# Autodesk Inventor assembly: Photosensor Assembly Exploded
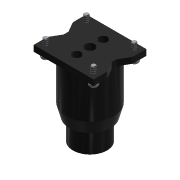
[picture p0: Inventor's stored thumbnail of the model, 180x180]
Saved by Autodesk Inventor 2017 (Build 210142000, 142)
## iProperties
Created: 2016-12-22
Part Number: Photosensor Assembly Exploded
Document SubType Name: Assembly
Designer: ge937963
Author: ge937963
## Documents named in this file (7)
- C:\Users\ge937963\Desktop\Inventor View\Photodiode Assembly.iam
- C:\Users\ge937963\Desktop\Inventor View\Photodiode Holder.ipt
- C:\Users\ge937963\Desktop\Inventor View\Emission Filter Holder.ipt
- C:\Users\ge937963\Desktop\Inventor View\Photodiode Assembly Mount.ipt
- C:\Users\ge937963\Desktop\Inventor View\Photodiode.ipt
- C:\Users\ge937963\Desktop\Inventor View\Screw.ipt
- C:\Users\ge937963\Desktop\Inventor View\Emission Filter.ipt
## Components (13 placed, 6 different names)
1. Photodiode Holder:1 — Mate:15, Mate:16, Mate:18
2. Emission Filter Holder:1 — Mate:18, Mate:19, Mate:21, Mate:22
3. Photodiode Assembly Mount:1 — Mate:16, Mate:20
4. Photodiode:1 — Mate:15
5. Screw:1 — Mate:20
6. Screw:2
7. Screw:3
8. Screw:4 — Mate:19
9. Screw:5
10. Screw:6
11. Screw:7
12. Screw:8
13. Emission Filter:1 — Mate:21, Mate:22
## Relationships (25: Mate 20, Flush 5)
- [Mate]: Photodiode Holder:1 ↔ Emission Filter Holder:1
- [Mate]: Photodiode Holder:1 ↔ Emission Filter Holder:1
- [Mate]: Photodiode Holder:1 ↔ Photodiode Assembly Mount:1
- [Mate]: Photodiode Holder:1 ↔ Photodiode Assembly Mount:1
- [Mate]: Photodiode Holder:1 ↔ Photodiode:1
- [Mate]: Emission Filter Holder:1 ↔ Screw:3
- [Mate]: Emission Filter Holder:1 ↔ Screw:4
- [Flush]: Screw:3 ↔ Screw:4
- [Flush]: Screw:1 ↔ Screw:2
- [Mate]: Photodiode Assembly Mount:1 ↔ Screw:1
- [Mate]: Photodiode Assembly Mount:1 ↔ Screw:2
- [Mate]: Photodiode Assembly Mount:1 ↔ Screw:5
- [Mate]: Photodiode Assembly Mount:1 ↔ Screw:6
- [Mate]: Photodiode Assembly Mount:1 ↔ Screw:7
- [Mate]: Photodiode Assembly Mount:1 ↔ Screw:8
- [Flush]: Screw:7 ↔ Screw:8
- [Flush]: Screw:5 ↔ Screw:6
- [Flush]: Screw:6 ↔ Screw:7
- Mate:15: Photodiode Holder:1 ↔ Photodiode:1
- Mate:16: Photodiode Holder:1 ↔ Photodiode Assembly Mount:1
- Mate:18: Photodiode Holder:1 ↔ Emission Filter Holder:1
- Mate:19: Emission Filter Holder:1 ↔ Screw:4
- Mate:20: Photodiode Assembly Mount:1 ↔ Screw:1
- Mate:21: Emission Filter Holder:1 ↔ Emission Filter:1
- Mate:22: Emission Filter Holder:1 ↔ Emission Filter:1
